# Autodesk Inventor assembly: Montagem_Tanque
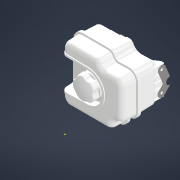
[picture p0: Inventor's stored thumbnail of the model, 180x180]
Saved by Autodesk Inventor 2022 (Build 260153000, 153)
## iProperties
Created: 2022-05-20
Part Number: Montagem_Tanque
Document SubType Name: Assembly
Designer: Gugarauj07
Author: Gugarauj07
## Documents named in this file (4)
- C:\Users\Gugarauj07\PycharmProjects\Eletronica_2022\CADS\Montagem_Tanque.iam
- C:\Users\Gugarauj07\PycharmProjects\Eletronica_2022\CADS\Gas Tank.ipt
- C:\Users\Gugarauj07\PycharmProjects\Eletronica_2022\CADS\FixaçãoTanque_1.ipt
- C:\Users\Gugarauj07\PycharmProjects\Eletronica_2022\CADS\FixaçãoTanque_2.ipt
## Components (3 placed, 3 different names)
1. Gas Tank:1 — Inserir:1, Inserir:2, Inserir:3, Inserir:4, Inserir:5
2. FixaçãoTanque_1:1 — Inserir:1, Inserir:2, Inserir:3
3. FixaçãoTanque_2:1 — Inserir:4, Inserir:5
## Relationships (5: Insert 5)
- Inserir:1: Gas Tank:1 ↔ FixaçãoTanque_1:1
- Inserir:2: Gas Tank:1 ↔ FixaçãoTanque_1:1
- Inserir:3 (50.8 mm): Gas Tank:1 ↔ FixaçãoTanque_1:1
- Inserir:4: Gas Tank:1 ↔ FixaçãoTanque_2:1
- Inserir:5: Gas Tank:1 ↔ FixaçãoTanque_2:1
